# Autodesk Inventor assembly: Piston Build Platform assy
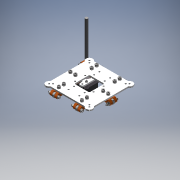
[picture p0: Inventor's stored thumbnail of the model, 180x180]
Saved by Autodesk Inventor 2018 (Build 220112000, 112)
## iProperties
Created: 2017-09-27
Part Number: Piston Build Platform assy
Document SubType Name: Assembly
Designer: Gabriel Smolnycki
Author: Gabriel Smolnycki
## Documents named in this file (7)
- H:\dev\planb\mechanics\V1INV\Subassemblies\Piston Build Platform assy.iam
- H:\dev\planb\mechanics\V1INV\Piston\Piston Build Frame.ipt
- H:\dev\planb\mechanics\V1INV\Subassemblies\Piston Wall Guide assy.iam
- H:\dev\planb\mechanics\V1INV\Hardware\M4 SS Washer.ipt
- H:\dev\planb\mechanics\V1INV\Hardware\M4 SS Locknut.ipt
- H:\dev\planb\mechanics\V1INV\Hardware\M4x25 SS SHCS.ipt
- H:\dev\planb\mechanics\V1INV\Subassemblies\Piston Motor Holder assy.iam
## Components (56 placed, 6 different names)
1. Piston Build Frame:1 — Insert:1, Insert:2, Insert:3, Insert:4, Insert:5, Insert:6, Insert:7, Insert:8, Insert:9, Insert:10, Insert:11, Insert:12, Insert:13, Insert:14, Insert:15, Insert:16, Insert:17, Insert:18, Insert:19, Insert:20, Insert:21, Insert:22, Insert:23, Insert:24
2. Piston Wall Guide assy:1 [sub-assembly] — Insert:1, Insert:2, Insert:27, Insert:28
3. Piston Wall Guide assy:2 [sub-assembly] — Insert:3, Insert:4, Insert:25, Insert:26
4. Piston Wall Guide assy:3 [sub-assembly] — Insert:7, Insert:8, Insert:31, Insert:32
5. Piston Wall Guide assy:4 [sub-assembly] — Insert:5, Insert:6, Insert:29, Insert:30
6. Piston Wall Guide assy:5 [sub-assembly] — Insert:11, Insert:12, Insert:35, Insert:36
7. Piston Wall Guide assy:6 [sub-assembly] — Insert:9, Insert:10, Insert:33, Insert:34
8. M4x25 SS SHCS:1
9. M4x25 SS SHCS:2
10. M4x25 SS SHCS:3
11. M4x25 SS SHCS:4
12. M4x25 SS SHCS:5
13. M4x25 SS SHCS:6
14. M4x25 SS SHCS:7
15. M4x25 SS SHCS:8
16. M4x25 SS SHCS:9
17. M4x25 SS SHCS:10
18. M4x25 SS SHCS:11
19. M4x25 SS SHCS:12
20. M4 SS Washer:1 — Insert:14
21. M4 SS Washer:2 — Insert:16
22. M4 SS Washer:3 — Insert:21
23. M4 SS Washer:4 — Insert:22
24. M4 SS Washer:5 — Insert:13
25. M4 SS Washer:6 — Insert:17
26. M4 SS Washer:7 — Insert:20
27. M4 SS Washer:8 — Insert:36, Insert:48
28. M4 SS Washer:9 — Insert:15
29. M4 SS Washer:10 — Insert:18
30. M4 SS Washer:11 — Insert:19
31. M4 SS Washer:12 — Insert:23
32. M4 SS Washer:13 — Insert:32, Insert:44
33. M4 SS Washer:14 — Insert:31, Insert:43
34. M4 SS Washer:15 — Insert:30, Insert:39
35. M4 SS Washer:16 — Insert:29, Insert:40
36. M4 SS Washer:17 — Insert:35, Insert:47
37. M4 SS Washer:18 — Insert:34, Insert:46
38. M4 SS Washer:19 — Insert:33, Insert:45
39. M4 SS Washer:20 — Insert:28, Insert:42
40. M4 SS Washer:21 — Insert:24
41. M4 SS Washer:22 — Insert:27, Insert:41
42. M4 SS Washer:23 — Insert:26, Insert:38
43. M4 SS Washer:24 — Insert:25, Insert:37
44. M4 SS Locknut:1 — Insert:46
45. M4 SS Locknut:2 — Insert:45
46. M4 SS Locknut:3 — Insert:43
47. M4 SS Locknut:4 — Insert:41
48. M4 SS Locknut:5 — Insert:39
49. M4 SS Locknut:6 — Insert:37
50. M4 SS Locknut:7 — Insert:48
51. M4 SS Locknut:8 — Insert:47
52. M4 SS Locknut:9 — Insert:44
53. M4 SS Locknut:10 — Insert:42
54. M4 SS Locknut:11 — Insert:40
55. M4 SS Locknut:12 — Insert:38
56. Piston Motor Holder assy:1 [sub-assembly]
## Relationships (60: Insert 60)
- Insert:1: Piston Build Frame:1 ↔ Piston Wall Guide assy:1
- Insert:2: Piston Build Frame:1 ↔ Piston Wall Guide assy:1
- Insert:3: Piston Build Frame:1 ↔ Piston Wall Guide assy:2
- Insert:4: Piston Build Frame:1 ↔ Piston Wall Guide assy:2
- Insert:5: Piston Build Frame:1 ↔ Piston Wall Guide assy:4
- Insert:6: Piston Build Frame:1 ↔ Piston Wall Guide assy:4
- Insert:7: Piston Build Frame:1 ↔ Piston Wall Guide assy:3
- Insert:8: Piston Build Frame:1 ↔ Piston Wall Guide assy:3
- Insert:9: Piston Build Frame:1 ↔ Piston Wall Guide assy:6
- Insert:10: Piston Build Frame:1 ↔ Piston Wall Guide assy:6
- Insert:11: Piston Build Frame:1 ↔ Piston Wall Guide assy:5
- Insert:12: Piston Build Frame:1 ↔ Piston Wall Guide assy:5
- Insert:13: Piston Build Frame:1 ↔ M4 SS Washer:5
- Insert:14: Piston Build Frame:1 ↔ M4 SS Washer:1
- Insert:15: Piston Build Frame:1 ↔ M4 SS Washer:9
- Insert:16: Piston Build Frame:1 ↔ M4 SS Washer:2
- Insert:17: Piston Build Frame:1 ↔ M4 SS Washer:6
- Insert:18: Piston Build Frame:1 ↔ M4 SS Washer:10
- Insert:19: Piston Build Frame:1 ↔ M4 SS Washer:11
- Insert:20: Piston Build Frame:1 ↔ M4 SS Washer:7
- Insert:21: Piston Build Frame:1 ↔ M4 SS Washer:3
- Insert:22: Piston Build Frame:1 ↔ M4 SS Washer:4
- Insert:23: Piston Build Frame:1 ↔ M4 SS Washer:12
- Insert:24: Piston Build Frame:1 ↔ M4 SS Washer:21
- Insert:25: Piston Wall Guide assy:2 ↔ M4 SS Washer:24
- Insert:26: Piston Wall Guide assy:2 ↔ M4 SS Washer:23
- Insert:27: Piston Wall Guide assy:1 ↔ M4 SS Washer:22
- Insert:28: Piston Wall Guide assy:1 ↔ M4 SS Washer:20
- Insert:29: Piston Wall Guide assy:4 ↔ M4 SS Washer:16
- Insert:30: Piston Wall Guide assy:4 ↔ M4 SS Washer:15
- Insert:31: Piston Wall Guide assy:3 ↔ M4 SS Washer:14
- Insert:32: Piston Wall Guide assy:3 ↔ M4 SS Washer:13
- Insert:33: Piston Wall Guide assy:6 ↔ M4 SS Washer:19
- Insert:34: Piston Wall Guide assy:6 ↔ M4 SS Washer:18
- Insert:35: Piston Wall Guide assy:5 ↔ M4 SS Washer:17
- Insert:36: Piston Wall Guide assy:5 ↔ M4 SS Washer:8
- Insert:37: M4 SS Washer:24 ↔ M4 SS Locknut:6
- Insert:38: M4 SS Washer:23 ↔ M4 SS Locknut:12
- Insert:39: M4 SS Washer:15 ↔ M4 SS Locknut:5
- Insert:40: M4 SS Washer:16 ↔ M4 SS Locknut:11
- Insert:41: M4 SS Washer:22 ↔ M4 SS Locknut:4
- Insert:42: M4 SS Washer:20 ↔ M4 SS Locknut:10
- Insert:43: M4 SS Washer:14 ↔ M4 SS Locknut:3
- Insert:44: M4 SS Washer:13 ↔ M4 SS Locknut:9
- Insert:45: M4 SS Washer:19 ↔ M4 SS Locknut:2
- Insert:46: M4 SS Washer:18 ↔ M4 SS Locknut:1
- Insert:47: M4 SS Washer:17 ↔ M4 SS Locknut:8
- Insert:48: M4 SS Washer:8 ↔ M4 SS Locknut:7
- [Insert]: M4x25 SS SHCS:12 ↔ M4 SS Washer:9
- [Insert]: M4x25 SS SHCS:11 ↔ M4 SS Washer:2
- [Insert]: M4x25 SS SHCS:3 ↔ M4 SS Washer:6
- [Insert]: M4x25 SS SHCS:4 ↔ M4 SS Washer:10
- [Insert]: M4x25 SS SHCS:5 ↔ M4 SS Washer:7
- [Insert]: M4x25 SS SHCS:6 ↔ M4 SS Washer:11
- [Insert]: M4x25 SS SHCS:9 ↔ M4 SS Washer:5
- [Insert]: M4x25 SS SHCS:10 ↔ M4 SS Washer:1
- [Insert]: M4x25 SS SHCS:1 ↔ M4 SS Washer:12
- [Insert]: M4x25 SS SHCS:2 ↔ M4 SS Washer:21
- [Insert]: M4x25 SS SHCS:7 ↔ M4 SS Washer:3
- [Insert]: M4x25 SS SHCS:8 ↔ M4 SS Washer:4
